# Autodesk Inventor assembly: Servo-Arm-38mm-Ball-Joint
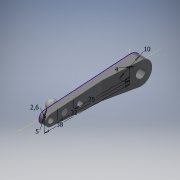
[picture p0: Inventor's stored thumbnail of the model, 180x180]
Saved by Autodesk Inventor 2018.2 (Build 222227000, 227)
## iProperties
Created: 2018-02-18
Part Number: Servo-Arm-38mm-Ball-Joint
Material: Generisch
Document SubType Name: Assembly
Designer: JochenAlt
Author: JochenAlt
## Documents named in this file (3)
- D:\Projects\Donna\CAD\KST DS215MG\Servo-Arm-38mm-Ball-Joint.iam
- D:\Projects\Donna\CAD\KST DS215MG\Servo-Arm-38mm.ipt
- D:\Projects\Donna\CAD\KST DS215MG\Ball-Joint-male.ipt
## Components (2 placed, 2 different names)
1. ServoArm:1 — Passend:3, Passend:5, Passend:6, Passend:8, Passend:9
2. ball joint:1 — Passend:3, Passend:9
## Relationships (5: Mate 5)
- Passend:3 [Mate]: ServoArm:1 ↔ ball joint:1
- Passend:5 [Mate]: ServoArm:1
- Passend:6 [Mate]: ServoArm:1
- Passend:8 [Mate]: ServoArm:1
- Passend:9 [Mate]: ServoArm:1 ↔ ball joint:1
